# Autodesk Inventor assembly: cellSTORM_v5_miniElectronics
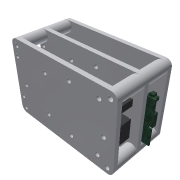
[picture p0: Inventor's stored thumbnail of the model, 180x180]
Saved by Autodesk Inventor 2019.4 (Build 234330000, 330)
## iProperties
Created: 2020-06-15
Part Number: cellSTORM_v5_miniElectronics
Document SubType Name: Assembly
Designer: diederichbenedict
Author: diederichbenedict
## Documents named in this file (6)
- C:\Users\diederichbenedict\Dropbox\Dokumente\Promotion\PROJECTS\STORMoChip\GITHUB\CAD\Nanoscopy-on-the-cheap\Workspace\cellSTORM_v5_miniElectronics.iam
- C:\Users\diederichbenedict\Dropbox\Dokumente\Promotion\PROJECTS\STORMoChip\GITHUB\CAD\Nanoscopy-on-the-cheap\Workspace\00_motordriver_pcb.ipt
- C:\Users\diederichbenedict\Dropbox\Dokumente\Promotion\PROJECTS\STORMoChip\GITHUB\CAD\Nanoscopy-on-the-cheap\Workspace\00_laserdriver_Pcb.ipt
- C:\Users\diederichbenedict\Dropbox\Dokumente\Promotion\PROJECTS\STORMoChip\GITHUB\CAD\Nanoscopy-on-the-cheap\Workspace\00_ESP32_Mini.ipt
- C:\Users\diederichbenedict\Dropbox\Dokumente\Promotion\PROJECTS\STORMoChip\GITHUB\CAD\Nanoscopy-on-the-cheap\Workspace\cellSTORM_v5_miniElectronics.ipt
- C:\Users\diederichbenedict\Dropbox\Dokumente\Promotion\PROJECTS\STORMoChip\GITHUB\CAD\Nanoscopy-on-the-cheap\Workspace\cellSTORM_v5_miniElectronics_lid.ipt
## Components (6 placed, 5 different names)
1. 00_motordriver_pcb:1 — Mate:2, Angle:1
2. 00_laserdriver_Pcb:1 — Mate:1, Flush:1, Flush:2
3. 00_ESP32_Mini:1 — Mate:3
4. cellSTORM_v5_miniElectronics:1 — Mate:1, Flush:1, Flush:2, Insert:1, Insert:2
5. cellSTORM_v5_miniElectronics:2 — Insert:1, Insert:2, Mate:2, Angle:1, Mate:3, Flush:3
6. cellSTORM_v5_miniElectronics_lid:1 — Flush:3
## Relationships (9: Mate 3, Flush 3, Insert 2, Angle 1)
- Mate:1: 00_laserdriver_Pcb:1 ↔ cellSTORM_v5_miniElectronics:1
- Flush:1 (2 mm): 00_laserdriver_Pcb:1 ↔ cellSTORM_v5_miniElectronics:1
- Flush:2 (10 mm): 00_laserdriver_Pcb:1 ↔ cellSTORM_v5_miniElectronics:1
- Insert:1: cellSTORM_v5_miniElectronics:1 ↔ cellSTORM_v5_miniElectronics:2
- Insert:2: cellSTORM_v5_miniElectronics:1 ↔ cellSTORM_v5_miniElectronics:2
- Mate:2: 00_motordriver_pcb:1 ↔ cellSTORM_v5_miniElectronics:2
- Angle:1 (0 deg): 00_motordriver_pcb:1 ↔ cellSTORM_v5_miniElectronics:2
- Mate:3: 00_ESP32_Mini:1 ↔ cellSTORM_v5_miniElectronics:2
- Flush:3: cellSTORM_v5_miniElectronics:2 ↔ cellSTORM_v5_miniElectronics_lid:1
